# Autodesk Inventor assembly: mirror_jig_test
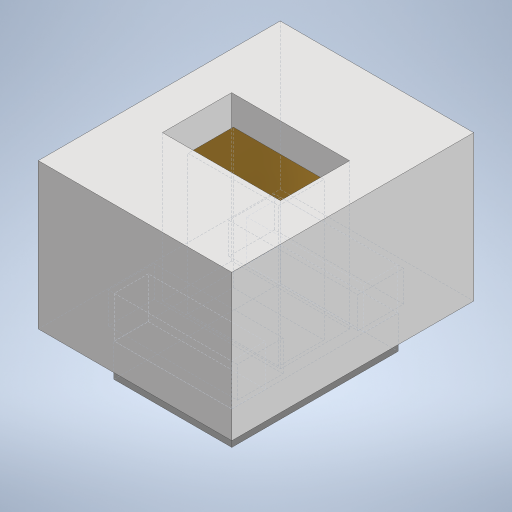
[picture p0: Inventor's stored thumbnail of the model, 512x512]
Saved by Autodesk Inventor 2023 (Build 270158000, 158)
## iProperties
Created: 2023-04-11
Part Number: mirror_jig_test
Document SubType Name: Assembly
Designer: Sam
Author: Sam
## Documents named in this file (3)
- C:\Users\Sam\Desktop\Glasspin\mirror_jig_test.iam
- C:\Users\Sam\Desktop\Glasspin\mirror_with_magnets.iam
- C:\Users\Sam\Desktop\Glasspin\magnet_jig.ipt
## Components (2 placed, 2 different names)
1. mirror_with_magnets:1 [sub-assembly] — Mate:3
2. magnet_jig:1 — Mate:1, Mate:2, Mate:3
## Relationships (3: Mate 3)
- Mate:1: magnet_jig:1
- Mate:2: magnet_jig:1
- Mate:3 (-2.6099 mm): mirror_with_magnets:1 ↔ magnet_jig:1
